# Autodesk Inventor assembly: crankshaft
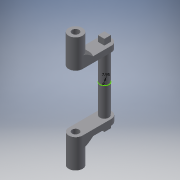
[picture p0: Inventor's stored thumbnail of the model, 180x180]
Saved by Autodesk Inventor 2018 (Build 220112000, 112)
## iProperties
Created: 2026-05-02
Part Number: crankshaft
Document SubType Name: Assembly
Designer: neo
Author: neo
## Documents named in this file (3)
- C:\Users\neo\Documents\projects\kreion\design2\crankshaft.iam
- C:\Users\neo\Documents\projects\kreion\design2\crankshaft_bearing_mounts.ipt
- C:\Users\neo\Documents\projects\kreion\design2\crankshaft_support.ipt
## Components (3 placed, 2 different names)
1. crankshaft_bearing_mounts:1 — Mate:1, Mate:2, Mate:3, Mate:4, Mate:5, Mate:6
2. crankshaft_support:1 — Mate:1, Mate:2, Mate:3
3. crankshaft_support:2 — Mate:4, Mate:5, Mate:6
## Relationships (6: Mate 6)
- Mate:1: crankshaft_bearing_mounts:1 ↔ crankshaft_support:1
- Mate:2: crankshaft_bearing_mounts:1 ↔ crankshaft_support:1
- Mate:3: crankshaft_bearing_mounts:1 ↔ crankshaft_support:1
- Mate:4: crankshaft_bearing_mounts:1 ↔ crankshaft_support:2
- Mate:5: crankshaft_bearing_mounts:1 ↔ crankshaft_support:2
- Mate:6: crankshaft_bearing_mounts:1 ↔ crankshaft_support:2
